# Autodesk Inventor assembly: CT4x4
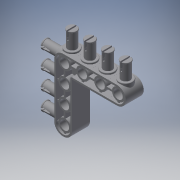
[picture p0: Inventor's stored thumbnail of the model, 180x180]
Saved by Autodesk Inventor 2019.3 (Build 233278000, 278)
## iProperties
Created: 2019-01-31
Part Number: CT4x4
Document SubType Name: Assembly
Designer: Varga Daniel
Vertical_hole_count: 4,000 ul
Horizontal_hole_count: 4,000 ul
Author: Varga Daniel
## Documents named in this file (11)
- C:\!_Dani\!_cloud\OneDrive\!_munka\Revolution\RevvyDemoKit\Structural parts\Connector Boxes\Connector triangle\CT2+x2+.iam
- C:\!_Dani\!_cloud\OneDrive\!_munka\Revolution\RevvyDemoKit\Structural parts\Beams\beam_single_end_part.ipt
- C:\!_Dani\!_cloud\OneDrive\!_munka\Revolution\RevvyDemoKit\Structural parts\Beams\beam_single_inner_part.ipt
- C:\!_Dani\!_cloud\OneDrive\!_munka\Revolution\RevvyDemoKit\Structural parts\Connetor Pins\Connector_pin_stick.ipt
- C:\!_Dani\!_cloud\OneDrive\!_munka\Revolution\RevvyDemoKit\Structural parts\Connector Boxes\Connector_box_L_base.ipt
- C:\!_Dani\!_cloud\OneDrive\!_munka\Revolution\RevvyDemoKit\Structural parts\Connector Boxes\Connector_box_collar\Connector_box_collar-one_side.ipt
- C:\!_Dani\!_cloud\OneDrive\!_munka\Revolution\RevvyDemoKit\Structural parts\Connector Boxes\Connector_box_collar.ipt
- C:\!_Dani\!_cloud\OneDrive\!_munka\Revolution\RevvyDemoKit\Structural parts\Connector Boxes\Connector_box_collar\Connector_box_collar-None.ipt
- CT2x2.iam
- CT3x3.iam
- CT4x4.iam
## Components (23 placed, 6 different names)
1. beam_single_end_part:1 — Flush:8, Flush:9, Mate:17, Mate:37, Mate:38, Mate:39, Angle:4
2. beam_single_end_part:2 — Mate:16, Flush:6, Flush:7, Mate:28, Mate:29, Angle:1, Mate:36
3. Connector_box_L_base:1 — Flush:1, Flush:2, Flush:3, Mate:14, Flush:4, Flush:5, Mate:15, Mate:16, Flush:6, Flush:7, Flush:8, Flush:9, Mate:17, Mate:40, Mate:41, Mate:42, Angle:5, Mate:43, Mate:44, Mate:45, Angle:6
4. Connector_box_collar-one_side:1 — Mate:18, Mate:19, Mate:37, Mate:38
5. Connector_pin_stick:2 — Mate:18, Mate:19, Mate:39, Angle:4
6. Connector_box_collar-one_side:3 — Mate:44, Mate:45
7. Connector_pin_stick:3 — Mate:43, Angle:6
8. Connector_box_collar-one_side:4 — Mate:41, Mate:42
9. Connector_pin_stick:4 — Mate:40, Angle:5
10. Connector_box_collar-one_side:5 — Mate:28, Mate:29
11. Connector_pin_stick:5 — Angle:1, Mate:36
12. beam_single_inner_part:2 — Flush:2, Mate:14, Flush:4, Flush:5, Mate:32, Mate:34, Angle:2
13. Connector_pin_stick:6 — Mate:34, Angle:2
14. Connector_box_collar-None:6 — Mate:32
15. beam_single_inner_part:3
16. Connector_pin_stick:7
17. Connector_box_collar-None:7
18. Connector_box_collar-None:2 — Mate:20, Mate:21, Mate:33
19. beam_single_inner_part:1 — Flush:1, Flush:3, Mate:15, Mate:33, Mate:35, Angle:3
20. Connector_pin_stick:1 — Mate:20, Mate:21, Mate:35, Angle:3
21. Connector_box_collar-None:8
22. beam_single_inner_part:4
23. Connector_pin_stick:8
## Component patterns: (2 elements, first: beam_single_inner_part:2 + Connector_pin_stick:6 + Connector_box_collar-None:6), (2 elements, first: Connector_box_collar-None:2 + beam_single_inner_part:1 + Connector_pin_stick:1)
## Relationships (47: Mate 32, Flush 9, Angle 6)
- Flush:1: Connector_box_L_base:1 ↔ beam_single_inner_part:1
- Flush:2: Connector_box_L_base:1 ↔ beam_single_inner_part:2
- Flush:3: Connector_box_L_base:1 ↔ beam_single_inner_part:1
- Mate:14: Connector_box_L_base:1 ↔ beam_single_inner_part:2
- Flush:4: Connector_box_L_base:1 ↔ beam_single_inner_part:2
- Flush:5: Connector_box_L_base:1 ↔ beam_single_inner_part:2
- Mate:15: Connector_box_L_base:1 ↔ beam_single_inner_part:1
- Mate:16 (20 mm): beam_single_end_part:2 ↔ Connector_box_L_base:1
- Flush:6: beam_single_end_part:2 ↔ Connector_box_L_base:1
- Flush:7: beam_single_end_part:2 ↔ Connector_box_L_base:1
- Flush:8: beam_single_end_part:1 ↔ Connector_box_L_base:1
- Flush:9: beam_single_end_part:1 ↔ Connector_box_L_base:1
- Mate:17 (20 mm): beam_single_end_part:1 ↔ Connector_box_L_base:1
- Mate:18: Connector_box_collar-one_side:1 ↔ Connector_pin_stick:2
- Mate:19: Connector_box_collar-one_side:1 ↔ Connector_pin_stick:2
- Mate:20: Connector_box_collar-None:2 ↔ Connector_pin_stick:1
- Mate:21: Connector_box_collar-None:2 ↔ Connector_pin_stick:1
- [Mate]: Connector_box_collar-one_side:3 ↔ Connector_pin_stick:3
- [Mate]: Connector_box_collar-one_side:3 ↔ Connector_pin_stick:3
- [Mate]: Connector_box_collar-one_side:4 ↔ Connector_pin_stick:4
- [Mate]: Connector_box_collar-one_side:4 ↔ Connector_pin_stick:4
- [Mate]: Connector_box_collar-one_side:5 ↔ Connector_pin_stick:5
- [Mate]: Connector_box_collar-one_side:5 ↔ Connector_pin_stick:5
- Mate:28: beam_single_end_part:2 ↔ Connector_box_collar-one_side:5
- Mate:29: beam_single_end_part:2 ↔ Connector_box_collar-one_side:5
- Angle:1 (0 deg): beam_single_end_part:2 ↔ Connector_pin_stick:5
- [Mate]: Connector_pin_stick:6 ↔ Connector_box_collar-None:6
- [Mate]: Connector_pin_stick:6 ↔ Connector_box_collar-None:6
- Mate:32: beam_single_inner_part:2 ↔ Connector_box_collar-None:6
- Mate:33: Connector_box_collar-None:2 ↔ beam_single_inner_part:1
- Mate:34: beam_single_inner_part:2 ↔ Connector_pin_stick:6
- Angle:2 (0 deg): beam_single_inner_part:2 ↔ Connector_pin_stick:6
- Mate:35: beam_single_inner_part:1 ↔ Connector_pin_stick:1
- Angle:3 (0 deg): beam_single_inner_part:1 ↔ Connector_pin_stick:1
- Mate:36: beam_single_end_part:2 ↔ Connector_pin_stick:5
- Mate:37: beam_single_end_part:1 ↔ Connector_box_collar-one_side:1
- Mate:38: beam_single_end_part:1 ↔ Connector_box_collar-one_side:1
- Mate:39: beam_single_end_part:1 ↔ Connector_pin_stick:2
- Angle:4 (0 deg): beam_single_end_part:1 ↔ Connector_pin_stick:2
- Mate:40: Connector_box_L_base:1 ↔ Connector_pin_stick:4
- Mate:41: Connector_box_L_base:1 ↔ Connector_box_collar-one_side:4
- Mate:42: Connector_box_L_base:1 ↔ Connector_box_collar-one_side:4
- Angle:5 (0 deg): Connector_box_L_base:1 ↔ Connector_pin_stick:4
- Mate:43: Connector_box_L_base:1 ↔ Connector_pin_stick:3
- Mate:44: Connector_box_L_base:1 ↔ Connector_box_collar-one_side:3
- Mate:45: Connector_box_L_base:1 ↔ Connector_box_collar-one_side:3
- Angle:6 (0 deg): Connector_box_L_base:1 ↔ Connector_pin_stick:3
## Named parameters: Vertical_hole_count = 4, Horizontal_hole_count = 4, d53_d49 = 0 mm, d54_d50 = 0 mm, d55_d49 = 0 mm, d56_d50 = 0 mm, d57_d49 = 0 mm, d58_d50 = 0 mm, d62_d51 = 0 mm, d63_d52 = 0 mm
